# Autodesk Inventor assembly: 弹舱
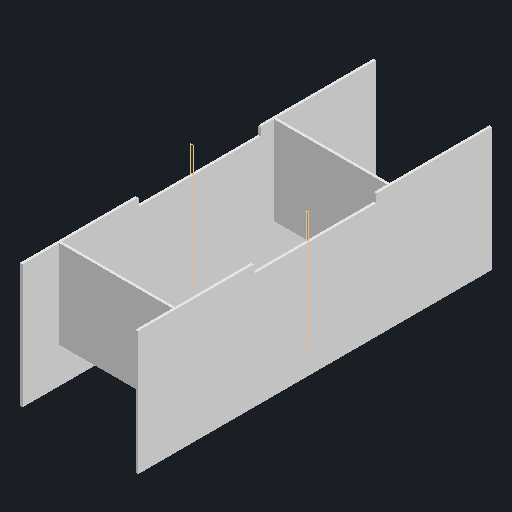
[picture p0: Inventor's stored thumbnail of the model, 512x512]
Saved by Autodesk Inventor 2025 (Build 290162000, 162)
## iProperties
Created: 2025-12-21
Part Number: 弹舱
Document SubType Name: Assembly
Designer: XH
Author: XH
## Documents named in this file (3)
- C:\1A_Engineering_files\RCInventor\铝件版本\板材料\玻纤\弹舱.iam
- C:\1A_Engineering_files\RCInventor\铝件版本\板材料\玻纤\弹舱1.ipt
- C:\1A_Engineering_files\RCInventor\铝件版本\板材料\玻纤\弹舱2.ipt
## Components (4 placed, 2 different names)
1. 弹舱1:1 — 表面齐平:1, 配合:1, 配合:2, 表面齐平:4
2. 弹舱2:1 — 表面齐平:1, 配合:1, 配合:3
3. 弹舱2:2 — 配合:2, 表面齐平:4, 表面齐平:5
4. 弹舱1:2 — 配合:3, 表面齐平:5
## Relationships (6: Flush 3, Mate 3)
- 表面齐平:1 [Flush]: 弹舱1:1 ↔ 弹舱2:1
- 配合:1 [Mate]: 弹舱1:1 ↔ 弹舱2:1
- 配合:2 [Mate]: 弹舱1:1 ↔ 弹舱2:2
- 表面齐平:4 [Flush]: 弹舱1:1 ↔ 弹舱2:2
- 配合:3 [Mate]: 弹舱2:1 ↔ 弹舱1:2
- 表面齐平:5 [Flush]: 弹舱2:2 ↔ 弹舱1:2
